# Autodesk Inventor assembly: ABB-IRB-120
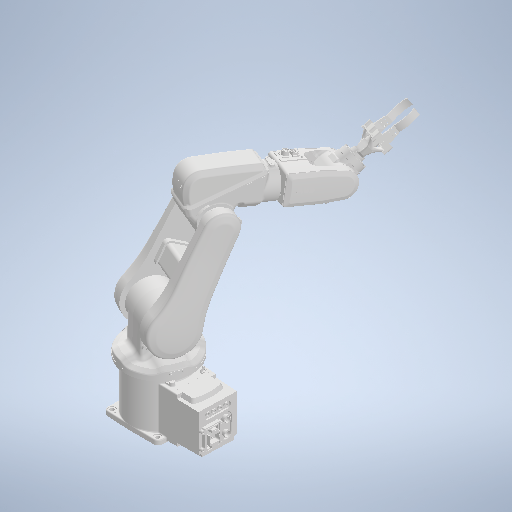
[picture p0: Inventor's stored thumbnail of the model, 512x512]
Saved by Autodesk Inventor 2025.1 (Build 291241000, 241)
## iProperties
Created: 2024-08-02
Part Number: ABB-IRB-120
Document SubType Name: Assembly
Designer: leonh
Author: leonh
## Documents named in this file (9)
- C:\Users\leonh\OneDrive\Dokumente\a_informatik\Inventor\Random\ABB-IRB-120.iam
- C:\Users\leonh\Downloads\rds-3225-servo-1.snapshot.1\RDS3225\STEP\IRB120_3-58_IRC5_Base_rev1\IRB120_3-58_IRC5_Base_rev1.iam
- C:\Users\leonh\Downloads\rds-3225-servo-1.snapshot.1\RDS3225\STEP\IRB120_3-58_IRC5_Link1_rev1\IRB120_3-58_IRC5_Link1_rev1.iam
- C:\Users\leonh\Downloads\rds-3225-servo-1.snapshot.1\RDS3225\STEP\IRB120_3-58_IRC5_Link2_rev1\IRB120_3-58_IRC5_Link2_rev1.iam
- C:\Users\leonh\Downloads\rds-3225-servo-1.snapshot.1\RDS3225\STEP\IRB120_3-58_IRC5_Link3_rev1\IRB120_3-58_IRC5_Link3_rev1.iam
- C:\Users\leonh\Downloads\rds-3225-servo-1.snapshot.1\RDS3225\STEP\IRB120_3-58_IRC5_Link4_rev1\IRB120_3-58_IRC5_Link4_rev1.iam
- C:\Users\leonh\Downloads\rds-3225-servo-1.snapshot.1\RDS3225\STEP\IRB120_3-58_IRC5_Link5_rev1\IRB120_3-58_IRC5_Link5_rev1.iam
- C:\Users\leonh\Downloads\rds-3225-servo-1.snapshot.1\RDS3225\STEP\IRB120_3-58_IRC5_Link6_rev1\IRB120_3-58_IRC5_Link6_rev1.ipt
- C:\Users\leonh\OneDrive\Dokumente\a_informatik\Inventor\Random\Gripper_Long_Assembly.iam
## Components (8 placed, 8 different names)
1. IRB120_3-58_IRC5_Base_rev1:1 [sub-assembly] — Rotational:1, Mate:1, Mate:2
2. IRB120_3-58_IRC5_Link1_rev1:1 [sub-assembly] — Rotational:1, Rotational:2
3. IRB120_3-58_IRC5_Link2_rev1:1 [sub-assembly] — Rotational:2, Rotational:3
4. IRB120_3-58_IRC5_Link3_rev1:1 [sub-assembly] — Rotational:3, Rotational:4
5. IRB120_3-58_IRC5_Link4_rev1:1 [sub-assembly] — Rotational:4, Rotational:5
6. IRB120_3-58_IRC5_Link5_rev1:1 [sub-assembly] — Rotational:5, Rotational:6
7. IRB120_3-58_IRC5_Link6_rev1:1 — Rotational:6, Mate:3, Mate:4, Angle:1
8. Gripper_Long_Assembly:1 [sub-assembly] — Mate:3, Mate:4, Angle:1
## Relationships (11: RevoluteJoint 6, Mate 4, Angle 1)
- Rotational:1 [RevoluteJoint]: IRB120_3-58_IRC5_Base_rev1:1 ↔ IRB120_3-58_IRC5_Link1_rev1:1
- Rotational:2 [RevoluteJoint]: IRB120_3-58_IRC5_Link1_rev1:1 ↔ IRB120_3-58_IRC5_Link2_rev1:1
- Rotational:3 [RevoluteJoint]: IRB120_3-58_IRC5_Link2_rev1:1 ↔ IRB120_3-58_IRC5_Link3_rev1:1
- Rotational:4 [RevoluteJoint]: IRB120_3-58_IRC5_Link3_rev1:1 ↔ IRB120_3-58_IRC5_Link4_rev1:1
- Rotational:5 [RevoluteJoint]: IRB120_3-58_IRC5_Link4_rev1:1 ↔ IRB120_3-58_IRC5_Link5_rev1:1
- Rotational:6 [RevoluteJoint]: IRB120_3-58_IRC5_Link5_rev1:1 ↔ IRB120_3-58_IRC5_Link6_rev1:1
- Mate:1: IRB120_3-58_IRC5_Base_rev1:1
- Mate:2: IRB120_3-58_IRC5_Base_rev1:1
- Mate:3: IRB120_3-58_IRC5_Link6_rev1:1 ↔ Gripper_Long_Assembly:1
- Mate:4: IRB120_3-58_IRC5_Link6_rev1:1 ↔ Gripper_Long_Assembly:1
- Angle:1 (180 deg): IRB120_3-58_IRC5_Link6_rev1:1 ↔ Gripper_Long_Assembly:1
